# Autodesk Inventor assembly: SSCSW12-10
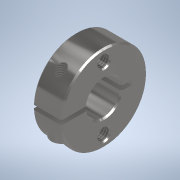
[picture p0: Inventor's stored thumbnail of the model, 180x180]
Saved by Autodesk Inventor 2021 (Build 250183000, 183)
## iProperties
Part Number: SSCSW12-10
Catalog Web Link: www.cadenas.de
Description: SCSW, PSCSW, SSCSW-Shaft Collars - 2-Tapped (Coarse Thread)
Vendor: MISUMI
Document SubType Name: Assembly
Designer: partserver
Manufacturer: MISUMI
Mass: 5.31236 g
Surface Area: 33.6487 cm^2
Volume: 5.31236 cm^3
Density: 1 g/cm^3
Category: PARTsolutions
Company: MISUMI
PSOL_IDENT_0: {$CADENAS_DATA\23d-libs\misumi\metric\03_set_collars\scsw_asmtab.prj},197 {VTYP=3D},{STYP=ASSTAB},{N
PSOL_IDENT_1: B=SSCSW12-10},{LINA=SSCSW12-10},{NN=SCSW, PSCSW, SSCSW},{DATE=09.09.2019 15:26:50},{GEOMDATE=24.02.2
PSOL_IDENT_2: 016 04:35:42},{VERSION=},{LINEID=70},{WBVAR=MAT,ST,BS},{WBNUMERIC=BS}  {NB=SSCSW12-10},{LINA=SSCSW12
PSOL_IDENT_3: -10},{KT=DUMMY},{PN=SSCSW12-10},{TYPE=SSCSW},{MAT=304},{ST=-},{AC=Hexagon Socket Head Set Screw 1 Pc
PSOL_IDENT_4: . (304 Stainless Steel) },{D=12},{BS=10},{D1=30},{M=M4},{THMD=4},{THDMIN=3.242},{ST0='-','-'},{B1=8,
PSOL_IDENT_5: 10,12,15},{DD=4.5},{R=3.75},{W=1.5},{X=10.0},{Y=5.0},{Z=9~10},{S=5.5},{P=22},{C=0.5},{L=12},{M1=M5},
PSOL_IDENT_6: {ZZ=9.5},{THMD1=5},{THDMIN1=4.134},{PPATH=scsw_templ.prj}
NB: SSCSW12-10
NN: SCSW, PSCSW, SSCSW
NT: Shaft Collars - 2-Tapped (Coarse Thread)
NBSYN: $PN.
LINA: SSCSW12-10
CATALOG: Misumi
PN: SSCSW12-10
MAT: SUS304 Equivalent
ST: -
AC: Hexagon Socket Head Set Screw 1 Pc. (304 Stainless Steel)
D: 12
BS: 10
D1: 30
M: M4
DD: 4.5
R: 3.75
W: 1.5
X: 10
Y: 5
Z: 9~10
S: 5.5
P: 22
M1: M5
SUPPLIER: MISUMI
ARTICLENO: SSCSW12-10
BOMINFO: SSCSW12-10
CREATOR: CADENAS GmbH
Title: SSCSW12-10
Author: Cadenas PARTsolutions
Comments: Shaft Collars - 2-Tapped (Coarse Thread)
## Documents named in this file (3)
- C:\Users\Hagihara Yuya\Documents\Inventor\Projects\NHK2021\DoRa-Chan\SetColor\SetColor_SSCSW12-10\SSCSW12-10.iam
- C:\Users\Hagihara Yuya\Documents\Inventor\Projects\NHK2021\DoRa-Chan\SetColor\SetColor_SSCSW12-10\SSCSW12-10b.ipt
- C:\Users\Hagihara Yuya\Documents\Inventor\Projects\NHK2021\DoRa-Chan\SetColor\SetColor_SSCSW12-10\Slotted head cap screw ISO 4762 - M4x12.ipt
## Components (2 placed, 2 different names)
1. SSCSW12-10b:1 — body_screw_Z@1 <-> IP1_Z@2
2. Slotted head cap screw ISO 4762 - M4x12:1 — body_screw_Z@1 <-> IP1_Z@2
## Relationships (1: Mate 1)
- body_screw_Z@1 <-> IP1_Z@2 [Mate]: SSCSW12-10b:1 ↔ Slotted head cap screw ISO 4762 - M4x12:1
